# Autodesk Inventor assembly: Nexus 7 3D hologram complete
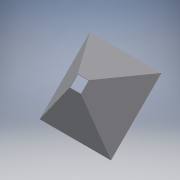
[picture p0: Inventor's stored thumbnail of the model, 180x180]
Saved by Autodesk Inventor 2016 (Build 200138000, 138)
## iProperties
Created: 2017-08-31
Part Number: Nexus 7 3D hologram complete
Document SubType Name: Assembly
Designer: student
Author: student
## Documents named in this file (2)
- C:\Users\student\Documents\Aaron's Folder\Nexus 7 3D hologram complete.iam
- C:\Users\student\Documents\Aaron's Folder\Nexus 7 3D hologram frame.ipt
## Components (4 placed, 1 different names)
1. Nexus 7 3D hologram frame:1 — Mate:1, Mate:2, Mate:3, Mate:7, Mate:8
2. Nexus 7 3D hologram frame:4 — Mate:1, Mate:2, Mate:3, Mate:4, Mate:5, Mate:6
3. Nexus 7 3D hologram frame:5 — Mate:4, Mate:5, Mate:6
4. Nexus 7 3D hologram frame:6 — Mate:7, Mate:8
## Relationships (8: Mate 8)
- Mate:1: Nexus 7 3D hologram frame:1 ↔ Nexus 7 3D hologram frame:4
- Mate:2: Nexus 7 3D hologram frame:1 ↔ Nexus 7 3D hologram frame:4
- Mate:3: Nexus 7 3D hologram frame:1 ↔ Nexus 7 3D hologram frame:4
- Mate:4: Nexus 7 3D hologram frame:4 ↔ Nexus 7 3D hologram frame:5
- Mate:5: Nexus 7 3D hologram frame:4 ↔ Nexus 7 3D hologram frame:5
- Mate:6: Nexus 7 3D hologram frame:4 ↔ Nexus 7 3D hologram frame:5
- Mate:7: Nexus 7 3D hologram frame:1 ↔ Nexus 7 3D hologram frame:6
- Mate:8: Nexus 7 3D hologram frame:1 ↔ Nexus 7 3D hologram frame:6
